# Autodesk Inventor assembly: ASSEMBLY_Main
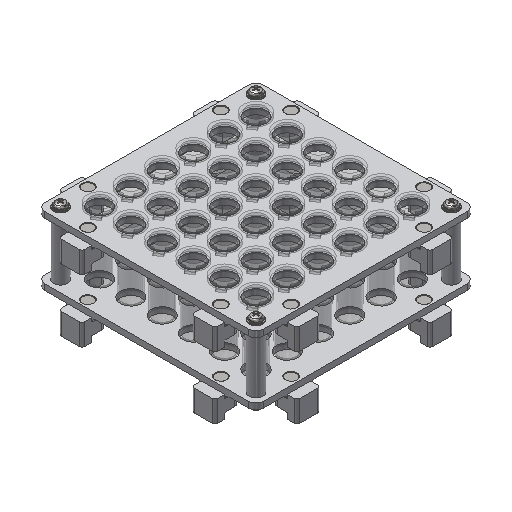
[picture p0: Inventor's stored thumbnail of the model, 512x512]
Saved by Autodesk Inventor 2025 (Build 290162010, 162A)
## iProperties
Created: 2018-06-17
Part Number: ASSEMBLY_Main
Document SubType Name: Assembly
Designer: Andrzej
Author: Andrzej
## Documents named in this file (8)
- D:\_ANDRZEJ_LACZEWSKI\_OTHER\MECH - SMD Parts Organizer\MCAD\1_REV1\ASSEMBLY_MAIN_REVA\ASSEMBLY_Main.iam
- D:\_ANDRZEJ_LACZEWSKI\_OTHER\MECH - SMD Parts Organizer\MCAD\1_REV1\__COTS_PARTS\COTS_Eppendorf_10ml_test_tube.ipt
- D:\_ANDRZEJ_LACZEWSKI\_OTHER\MECH - SMD Parts Organizer\MCAD\1_REV1\ASSEMBLY_MAIN_REVA\3DP_PLA_Test_Tube_Plate.ipt
- D:\_ANDRZEJ_LACZEWSKI\_OTHER\MECH - SMD Parts Organizer\MCAD\1_REV1\__COTS_PARTS\COTS_GENERIC_6x3mm_Cylindricial_Neodymium_Magnet.ipt
- D:\_ANDRZEJ_LACZEWSKI\_OTHER\MECH - SMD Parts Organizer\MCAD\1_REV1\ASSEMBLY_MAIN_REVA\3DP_PLA_Spacer.ipt
- D:\_ANDRZEJ_LACZEWSKI\_OTHER\MECH - SMD Parts Organizer\MCAD\1_REV1\__CONTENT_CENTER_PARTS\en-US\DIN 125-2  A\DIN 125-2 - A 3,2A.ipt
- D:\_ANDRZEJ_LACZEWSKI\_OTHER\MECH - SMD Parts Organizer\MCAD\1_REV1\__CONTENT_CENTER_PARTS\en-US\AS 1427(05)\AS 1427 - M3 x 40(5) II.ipt
- D:\_ANDRZEJ_LACZEWSKI\_OTHER\MECH - SMD Parts Organizer\MCAD\1_REV1\__CONTENT_CENTER_PARTS\en-US\DIN 934\DIN 934 - M3 x 0,5.ipt
## Components (90 placed, 7 different names)
1. 3DP_PLA_Spacer:1 — Mate:36, Mate:42
2. 3DP_PLA_Spacer:2 — Mate:37, Mate:43
3. 3DP_PLA_Spacer:3 — Mate:38, Mate:40
4. 3DP_PLA_Spacer:4 — Mate:39, Mate:41
5. DIN 125-2 A A 3,2:1 — Mate:44, Mate:45, Insert:1
6. AS 1427 H - Metric M3 x 40:1 — Insert:1
7. DIN 125-2 A A 3,2:2 — Mate:52, Mate:53, Insert:5
8. DIN 934 - replaced by DIN EN 24032/28673/28674 M3:1 — Insert:5
9. DIN 125-2 A A 3,2:3 — Mate:46, Mate:47, Insert:2
10. DIN 125-2 A A 3,2:4 — Mate:48, Mate:49, Insert:3
11. DIN 125-2 A A 3,2:5 — Mate:50, Mate:51, Insert:4
12. AS 1427 H - Metric M3 x 40:2 — Insert:2
13. AS 1427 H - Metric M3 x 40:3 — Insert:3
14. AS 1427 H - Metric M3 x 40:4 — Insert:4
15. DIN 125-2 A A 3,2:6 — Mate:54, Mate:55, Insert:6
16. DIN 125-2 A A 3,2:7 — Mate:56, Mate:57, Insert:7
17. DIN 125-2 A A 3,2:8 — Mate:58, Mate:59, Insert:8
18. DIN 934 - replaced by DIN EN 24032/28673/28674 M3:2 — Insert:6
19. DIN 934 - replaced by DIN EN 24032/28673/28674 M3:3 — Insert:7
20. DIN 934 - replaced by DIN EN 24032/28673/28674 M3:4 — Insert:8
21. COTS_Eppendorf_10ml_test_tube:1 — Mate:2, Mate:3
22. COTS_Eppendorf_10ml_test_tube:2
23. COTS_Eppendorf_10ml_test_tube:3
24. COTS_Eppendorf_10ml_test_tube:4
25. COTS_Eppendorf_10ml_test_tube:5
26. COTS_Eppendorf_10ml_test_tube:6
27. COTS_Eppendorf_10ml_test_tube:7
28. COTS_Eppendorf_10ml_test_tube:8
29. COTS_Eppendorf_10ml_test_tube:9
30. COTS_Eppendorf_10ml_test_tube:10
31. COTS_Eppendorf_10ml_test_tube:11
32. COTS_Eppendorf_10ml_test_tube:12
33. COTS_Eppendorf_10ml_test_tube:13
34. COTS_Eppendorf_10ml_test_tube:14
35. COTS_Eppendorf_10ml_test_tube:15
36. COTS_Eppendorf_10ml_test_tube:16
37. COTS_Eppendorf_10ml_test_tube:17
38. COTS_Eppendorf_10ml_test_tube:18
39. COTS_Eppendorf_10ml_test_tube:19
40. COTS_Eppendorf_10ml_test_tube:20
41. COTS_Eppendorf_10ml_test_tube:21
42. COTS_Eppendorf_10ml_test_tube:22
43. COTS_Eppendorf_10ml_test_tube:23
44. COTS_Eppendorf_10ml_test_tube:24
45. COTS_Eppendorf_10ml_test_tube:25
46. COTS_Eppendorf_10ml_test_tube:26
47. COTS_Eppendorf_10ml_test_tube:27
48. COTS_Eppendorf_10ml_test_tube:28
49. COTS_Eppendorf_10ml_test_tube:29
50. COTS_Eppendorf_10ml_test_tube:30
51. COTS_Eppendorf_10ml_test_tube:31
52. COTS_Eppendorf_10ml_test_tube:32
53. COTS_Eppendorf_10ml_test_tube:33
54. COTS_Eppendorf_10ml_test_tube:34
55. COTS_Eppendorf_10ml_test_tube:35
56. COTS_Eppendorf_10ml_test_tube:36
57. 3DP_PLA_Test_Tube_Plate:1 — Mate:2, Mate:3, Mate:4, Mate:5, Mate:6, Mate:7, Mate:8, Mate:9, Mate:10, Mate:11, Mate:12, Mate:13, Mate:14, Mate:15, Mate:16, Mate:17, Mate:18, Mate:19, Mate:20, Mate:21, Mate:22, Mate:23, Mate:24, Mate:25, Mate:26, Mate:27, Mate:28, Mate:29, Mate:30, Mate:31, Mate:32, Mate:33, Mate:34, Mate:35, Mate:44, Mate:45, Mate:46, Mate:47, Mate:48, Mate:49, Mate:50, Mate:51, Mate:52, Mate:54, Mate:56, Mate:58, Mate:60, Mate:61
58. COTS_GENERIC_6x3mm_Cylindricial_Neodymium_Magnet:1 — Mate:6, Mate:15
59. COTS_GENERIC_6x3mm_Cylindricial_Neodymium_Magnet:2 — Mate:11, Mate:12
60. COTS_GENERIC_6x3mm_Cylindricial_Neodymium_Magnet:3 — Mate:10, Mate:19
61. COTS_GENERIC_6x3mm_Cylindricial_Neodymium_Magnet:4 — Mate:9, Mate:18
62. COTS_GENERIC_6x3mm_Cylindricial_Neodymium_Magnet:5 — Mate:4, Mate:13
63. COTS_GENERIC_6x3mm_Cylindricial_Neodymium_Magnet:6 — Mate:5, Mate:14
64. COTS_GENERIC_6x3mm_Cylindricial_Neodymium_Magnet:7 — Mate:7, Mate:16
65. COTS_GENERIC_6x3mm_Cylindricial_Neodymium_Magnet:8 — Mate:8, Mate:17
66. COTS_GENERIC_6x3mm_Cylindricial_Neodymium_Magnet:9 — Mate:20, Mate:33
67. COTS_GENERIC_6x3mm_Cylindricial_Neodymium_Magnet:10 — Mate:21, Mate:34
68. COTS_GENERIC_6x3mm_Cylindricial_Neodymium_Magnet:11 — Mate:22, Mate:32
69. COTS_GENERIC_6x3mm_Cylindricial_Neodymium_Magnet:12 — Mate:23, Mate:31
70. COTS_GENERIC_6x3mm_Cylindricial_Neodymium_Magnet:13 — Mate:27, Mate:28
71. COTS_GENERIC_6x3mm_Cylindricial_Neodymium_Magnet:14 — Mate:26, Mate:35
72. COTS_GENERIC_6x3mm_Cylindricial_Neodymium_Magnet:15 — Mate:24, Mate:30
73. COTS_GENERIC_6x3mm_Cylindricial_Neodymium_Magnet:16 — Mate:25, Mate:29
74. 3DP_PLA_Test_Tube_Plate:2 — Mate:36, Mate:37, Mate:38, Mate:39, Mate:40, Mate:41, Mate:42, Mate:43, Mate:53, Mate:55, Mate:57, Mate:59
75. COTS_GENERIC_6x3mm_Cylindricial_Neodymium_Magnet:17
76. COTS_GENERIC_6x3mm_Cylindricial_Neodymium_Magnet:18
77. COTS_GENERIC_6x3mm_Cylindricial_Neodymium_Magnet:19
78. COTS_GENERIC_6x3mm_Cylindricial_Neodymium_Magnet:20
79. COTS_GENERIC_6x3mm_Cylindricial_Neodymium_Magnet:21
80. COTS_GENERIC_6x3mm_Cylindricial_Neodymium_Magnet:22
81. COTS_GENERIC_6x3mm_Cylindricial_Neodymium_Magnet:23
82. COTS_GENERIC_6x3mm_Cylindricial_Neodymium_Magnet:24
83. COTS_GENERIC_6x3mm_Cylindricial_Neodymium_Magnet:25
84. COTS_GENERIC_6x3mm_Cylindricial_Neodymium_Magnet:26
85. COTS_GENERIC_6x3mm_Cylindricial_Neodymium_Magnet:27
86. COTS_GENERIC_6x3mm_Cylindricial_Neodymium_Magnet:28
87. COTS_GENERIC_6x3mm_Cylindricial_Neodymium_Magnet:29
88. COTS_GENERIC_6x3mm_Cylindricial_Neodymium_Magnet:30
89. COTS_GENERIC_6x3mm_Cylindricial_Neodymium_Magnet:31
90. COTS_GENERIC_6x3mm_Cylindricial_Neodymium_Magnet:32
## Component patterns: (36 elements, first: COTS_Eppendorf_10ml_test_tube:1), (2 elements, first: 3DP_PLA_Test_Tube_Plate:1 + COTS_GENERIC_6x3mm_Cylindricial_Neodymium_Magnet:1 + COTS_GENERIC_6x3mm_Cylindricial_Neodymium_Magnet:2 + COTS_GENERIC_6x3mm_Cylindricial_Neodymium_Magnet:3 + COTS_GENERIC_6x3mm_Cylindricial_Neodymium_Magnet:4 + COTS_GENERIC_6x3mm_Cylindricial_Neodymium_Magnet:5 + COTS_GENERIC_6x3mm_Cylindricial_Neodymium_Magnet:6 + COTS_GENERIC_6x3mm_Cylindricial_Neodymium_Magnet:7 + COTS_GENERIC_6x3mm_Cylindricial_Neodymium_Magnet:8 + COTS_GENERIC_6x3mm_Cylindricial_Neodymium_Magnet:9 + COTS_GENERIC_6x3mm_Cylindricial_Neodymium_Magnet:10 + COTS_GENERIC_6x3mm_Cylindricial_Neodymium_Magnet:11 + COTS_GENERIC_6x3mm_Cylindricial_Neodymium_Magnet:12 + COTS_GENERIC_6x3mm_Cylindricial_Neodymium_Magnet:13 + COTS_GENERIC_6x3mm_Cylindricial_Neodymium_Magnet:14 + COTS_GENERIC_6x3mm_Cylindricial_Neodymium_Magnet:15 + COTS_GENERIC_6x3mm_Cylindricial_Neodymium_Magnet:16)
## Relationships (68: Mate 60, Insert 8)
- Mate:2: COTS_Eppendorf_10ml_test_tube:1 ↔ 3DP_PLA_Test_Tube_Plate:1
- Mate:3: COTS_Eppendorf_10ml_test_tube:1 ↔ 3DP_PLA_Test_Tube_Plate:1
- Mate:4: 3DP_PLA_Test_Tube_Plate:1 ↔ COTS_GENERIC_6x3mm_Cylindricial_Neodymium_Magnet:5
- Mate:5: 3DP_PLA_Test_Tube_Plate:1 ↔ COTS_GENERIC_6x3mm_Cylindricial_Neodymium_Magnet:6
- Mate:6: 3DP_PLA_Test_Tube_Plate:1 ↔ COTS_GENERIC_6x3mm_Cylindricial_Neodymium_Magnet:1
- Mate:7: 3DP_PLA_Test_Tube_Plate:1 ↔ COTS_GENERIC_6x3mm_Cylindricial_Neodymium_Magnet:7
- Mate:8: 3DP_PLA_Test_Tube_Plate:1 ↔ COTS_GENERIC_6x3mm_Cylindricial_Neodymium_Magnet:8
- Mate:9: 3DP_PLA_Test_Tube_Plate:1 ↔ COTS_GENERIC_6x3mm_Cylindricial_Neodymium_Magnet:4
- Mate:10: 3DP_PLA_Test_Tube_Plate:1 ↔ COTS_GENERIC_6x3mm_Cylindricial_Neodymium_Magnet:3
- Mate:11: 3DP_PLA_Test_Tube_Plate:1 ↔ COTS_GENERIC_6x3mm_Cylindricial_Neodymium_Magnet:2
- Mate:12: 3DP_PLA_Test_Tube_Plate:1 ↔ COTS_GENERIC_6x3mm_Cylindricial_Neodymium_Magnet:2
- Mate:13: 3DP_PLA_Test_Tube_Plate:1 ↔ COTS_GENERIC_6x3mm_Cylindricial_Neodymium_Magnet:5
- Mate:14: 3DP_PLA_Test_Tube_Plate:1 ↔ COTS_GENERIC_6x3mm_Cylindricial_Neodymium_Magnet:6
- Mate:15: 3DP_PLA_Test_Tube_Plate:1 ↔ COTS_GENERIC_6x3mm_Cylindricial_Neodymium_Magnet:1
- Mate:16: 3DP_PLA_Test_Tube_Plate:1 ↔ COTS_GENERIC_6x3mm_Cylindricial_Neodymium_Magnet:7
- Mate:17: 3DP_PLA_Test_Tube_Plate:1 ↔ COTS_GENERIC_6x3mm_Cylindricial_Neodymium_Magnet:8
- Mate:18: 3DP_PLA_Test_Tube_Plate:1 ↔ COTS_GENERIC_6x3mm_Cylindricial_Neodymium_Magnet:4
- Mate:19: 3DP_PLA_Test_Tube_Plate:1 ↔ COTS_GENERIC_6x3mm_Cylindricial_Neodymium_Magnet:3
- Mate:20: 3DP_PLA_Test_Tube_Plate:1 ↔ COTS_GENERIC_6x3mm_Cylindricial_Neodymium_Magnet:9
- Mate:21: 3DP_PLA_Test_Tube_Plate:1 ↔ COTS_GENERIC_6x3mm_Cylindricial_Neodymium_Magnet:10
- Mate:22: 3DP_PLA_Test_Tube_Plate:1 ↔ COTS_GENERIC_6x3mm_Cylindricial_Neodymium_Magnet:11
- Mate:23: 3DP_PLA_Test_Tube_Plate:1 ↔ COTS_GENERIC_6x3mm_Cylindricial_Neodymium_Magnet:12
- Mate:24: 3DP_PLA_Test_Tube_Plate:1 ↔ COTS_GENERIC_6x3mm_Cylindricial_Neodymium_Magnet:15
- Mate:25: 3DP_PLA_Test_Tube_Plate:1 ↔ COTS_GENERIC_6x3mm_Cylindricial_Neodymium_Magnet:16
- Mate:26: 3DP_PLA_Test_Tube_Plate:1 ↔ COTS_GENERIC_6x3mm_Cylindricial_Neodymium_Magnet:14
- Mate:27: 3DP_PLA_Test_Tube_Plate:1 ↔ COTS_GENERIC_6x3mm_Cylindricial_Neodymium_Magnet:13
- Mate:28: 3DP_PLA_Test_Tube_Plate:1 ↔ COTS_GENERIC_6x3mm_Cylindricial_Neodymium_Magnet:13
- Mate:29: 3DP_PLA_Test_Tube_Plate:1 ↔ COTS_GENERIC_6x3mm_Cylindricial_Neodymium_Magnet:16
- Mate:30: 3DP_PLA_Test_Tube_Plate:1 ↔ COTS_GENERIC_6x3mm_Cylindricial_Neodymium_Magnet:15
- Mate:31: 3DP_PLA_Test_Tube_Plate:1 ↔ COTS_GENERIC_6x3mm_Cylindricial_Neodymium_Magnet:12
- Mate:32: 3DP_PLA_Test_Tube_Plate:1 ↔ COTS_GENERIC_6x3mm_Cylindricial_Neodymium_Magnet:11
- Mate:33: 3DP_PLA_Test_Tube_Plate:1 ↔ COTS_GENERIC_6x3mm_Cylindricial_Neodymium_Magnet:9
- Mate:34: 3DP_PLA_Test_Tube_Plate:1 ↔ COTS_GENERIC_6x3mm_Cylindricial_Neodymium_Magnet:10
- Mate:35: 3DP_PLA_Test_Tube_Plate:1 ↔ COTS_GENERIC_6x3mm_Cylindricial_Neodymium_Magnet:14
- Mate:36: 3DP_PLA_Spacer:1 ↔ 3DP_PLA_Test_Tube_Plate:2
- Mate:37: 3DP_PLA_Spacer:2 ↔ 3DP_PLA_Test_Tube_Plate:2
- Mate:38: 3DP_PLA_Spacer:3 ↔ 3DP_PLA_Test_Tube_Plate:2
- Mate:39: 3DP_PLA_Spacer:4 ↔ 3DP_PLA_Test_Tube_Plate:2
- Mate:40: 3DP_PLA_Spacer:3 ↔ 3DP_PLA_Test_Tube_Plate:2
- Mate:41: 3DP_PLA_Spacer:4 ↔ 3DP_PLA_Test_Tube_Plate:2
- Mate:42: 3DP_PLA_Spacer:1 ↔ 3DP_PLA_Test_Tube_Plate:2
- Mate:43: 3DP_PLA_Spacer:2 ↔ 3DP_PLA_Test_Tube_Plate:2
- Mate:44: DIN 125-2 A A 3,2:1 ↔ 3DP_PLA_Test_Tube_Plate:1
- Mate:45: DIN 125-2 A A 3,2:1 ↔ 3DP_PLA_Test_Tube_Plate:1
- Mate:46: DIN 125-2 A A 3,2:3 ↔ 3DP_PLA_Test_Tube_Plate:1
- Mate:47: DIN 125-2 A A 3,2:3 ↔ 3DP_PLA_Test_Tube_Plate:1
- Mate:48: DIN 125-2 A A 3,2:4 ↔ 3DP_PLA_Test_Tube_Plate:1
- Mate:49: DIN 125-2 A A 3,2:4 ↔ 3DP_PLA_Test_Tube_Plate:1
- Mate:50: DIN 125-2 A A 3,2:5 ↔ 3DP_PLA_Test_Tube_Plate:1
- Mate:51: DIN 125-2 A A 3,2:5 ↔ 3DP_PLA_Test_Tube_Plate:1
- Insert:1: DIN 125-2 A A 3,2:1 ↔ AS 1427 H - Metric M3 x 40:1
- Insert:2: DIN 125-2 A A 3,2:3 ↔ AS 1427 H - Metric M3 x 40:2
- Insert:3: DIN 125-2 A A 3,2:4 ↔ AS 1427 H - Metric M3 x 40:3
- Insert:4: DIN 125-2 A A 3,2:5 ↔ AS 1427 H - Metric M3 x 40:4
- Mate:52: DIN 125-2 A A 3,2:2 ↔ 3DP_PLA_Test_Tube_Plate:1
- Mate:53: DIN 125-2 A A 3,2:2 ↔ 3DP_PLA_Test_Tube_Plate:2
- Mate:54: DIN 125-2 A A 3,2:6 ↔ 3DP_PLA_Test_Tube_Plate:1
- Mate:55: DIN 125-2 A A 3,2:6 ↔ 3DP_PLA_Test_Tube_Plate:2
- Mate:56: DIN 125-2 A A 3,2:7 ↔ 3DP_PLA_Test_Tube_Plate:1
- Mate:57: DIN 125-2 A A 3,2:7 ↔ 3DP_PLA_Test_Tube_Plate:2
- Mate:58: DIN 125-2 A A 3,2:8 ↔ 3DP_PLA_Test_Tube_Plate:1
- Mate:59: DIN 125-2 A A 3,2:8 ↔ 3DP_PLA_Test_Tube_Plate:2
- Insert:5: DIN 125-2 A A 3,2:2 ↔ DIN 934 - replaced by DIN EN 24032/28673/28674 M3:1
- Insert:6: DIN 125-2 A A 3,2:6 ↔ DIN 934 - replaced by DIN EN 24032/28673/28674 M3:2
- Insert:7: DIN 125-2 A A 3,2:7 ↔ DIN 934 - replaced by DIN EN 24032/28673/28674 M3:3
- Insert:8: DIN 125-2 A A 3,2:8 ↔ DIN 934 - replaced by DIN EN 24032/28673/28674 M3:4
- Mate:60 (-56 mm): 3DP_PLA_Test_Tube_Plate:1
- Mate:61 (-56 mm): 3DP_PLA_Test_Tube_Plate:1
